# Autodesk Inventor assembly: front_hings
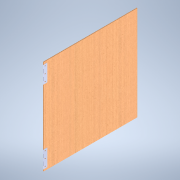
[picture p0: Inventor's stored thumbnail of the model, 180x180]
Saved by Autodesk Inventor 2020 (Build 240168000, 168)
## iProperties
Created: 2020-05-03
Part Number: front_hings
Document SubType Name: Assembly
Designer: galaxy
Author: galaxy
## Documents named in this file (3)
- C:\Users\galaxy\Desktop\control box\front_hings.iam
- C:\Users\galaxy\Desktop\control box\front_cover.ipt
- C:\Users\galaxy\Desktop\control box\Peice 2.ipt
## Components (3 placed, 2 different names)
1. front_cover:2 — Insert:1, Insert:2, Insert:3, Insert:4
2. Peice 2:1 — Insert:1, Insert:2
3. Peice 2:2 — Insert:3, Insert:4
## Relationships (4: Insert 4)
- Insert:1: front_cover:2 ↔ Peice 2:1
- Insert:2: front_cover:2 ↔ Peice 2:1
- Insert:3: front_cover:2 ↔ Peice 2:2
- Insert:4: front_cover:2 ↔ Peice 2:2
